# Autodesk Inventor assembly: s-assy-spacer2.ipt
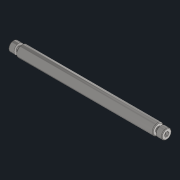
[picture p0: Inventor's stored thumbnail of the model, 180x180]
Saved by Autodesk Inventor 2021 (Build 250183000, 183)
## iProperties
Created: 2021-08-04
Part Number: s-assy-spacer2.ipt
Document SubType Name: Assembly
Designer: yuta0
Author: yuta0
## Documents named in this file (3)
- C:\Users\yuta0\Desktop\catchrobo_robot\s-assy-spacer2.ipt.iam
- C:\Users\yuta0\Desktop\catchrobo_robot\SFHRW8-98-M4-N4.ipt
- C:\Users\yuta0\Desktop\lab\nicebot\CB4-10.ipt
## Components (3 placed, 2 different names)
1. SFHRW8-98-M4-N4:1 — メイト:1, メイト:2, メイト:3, メイト:4
2. CB4-10:1 — メイト:1, メイト:4
3. CB4-10:2 — メイト:2, メイト:3
## Relationships (4: Mate 4)
- メイト:1 [Mate]: SFHRW8-98-M4-N4:1 ↔ CB4-10:1
- メイト:2 [Mate]: SFHRW8-98-M4-N4:1 ↔ CB4-10:2
- メイト:3 [Mate] (2 mm): SFHRW8-98-M4-N4:1 ↔ CB4-10:2
- メイト:4 [Mate] (2 mm): SFHRW8-98-M4-N4:1 ↔ CB4-10:1
